# Autodesk Inventor assembly: Refined Glock
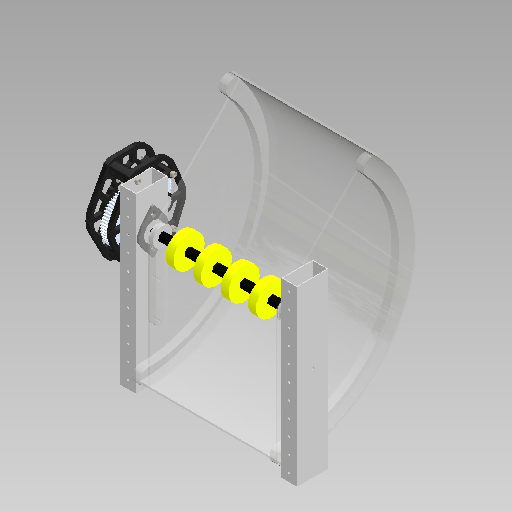
[picture p0: Inventor's stored thumbnail of the model, 512x512]
Saved by Autodesk Inventor 2021 (Build 250183000, 183)
## iProperties
Created: 2021-02-04
Part Number: Refined Glock
Document SubType Name: Assembly
Designer: aidan
Author: aidan
## Documents named in this file (12)
- C:\Users\Merkileg\Documents\t3-cad\CAD\2021 Specific Parts\Refined Glock.iam
- C:\Users\Merkileg\Documents\t3-cad\CAD\2021 Specific Parts\Curved Lexan Support.ipt
- C:\Users\Merkileg\Documents\t3-cad\CAD\2021 Specific Parts\Shooter side panel.ipt
- C:\Users\Merkileg\Documents\t3-cad\CAD\2021 Specific Parts\Lexan Glock Back.ipt
- C:\Users\Merkileg\Documents\t3-cad\CAD\Bearing for THUNDER.ipt
- C:\Users\Merkileg\Documents\t3-cad\CAD\WCP SS_Shrinkwrap.ipt
- C:\Users\Merkileg\Documents\t3-cad\CAD\2021 Specific Parts\VersaFrame Support for Glock.ipt
- C:\Users\Merkileg\Documents\t3-cad\CAD\Drive Train CAD\WCP DS Gearbox\WCP Gearbox Mount.ipt
- C:\Users\Merkileg\Documents\t3-cad\CAD\2021 Specific Parts\Side lexan spacer for Glock.ipt
- C:\Users\Merkileg\Documents\t3-cad\CAD\Generic and Stock\11.75in THUNDERSHAFT.ipt
- C:\Users\Merkileg\Documents\t3-cad\CAD\Tristan's CAD\Glock\2 in Compliance Wheel.ipt
- C:\Users\Merkileg\Documents\t3-cad\CAD\2021 Specific Parts\VerseFrame 11in w hole.ipt
## Components (19 placed, 11 different names)
1. Curved Lexan Support:1 — Mate:3, Mate:5, Mate:6, Mate:14
2. Curved Lexan Support:2 — Mate:3, Mate:4, Mate:5, Mate:7, Flush:3, Mate:9
3. Shooter side panel:1 — Flush:1, Flush:2, Mate:6, Mate:8, Mate:10, Mate:12, Angle:1, Mate:35
4. Shooter side panel:2 — Flush:1, Flush:2, Mate:4, Mate:7, Mate:8, Flush:4, Mate:11, Mate:13, Mate:30
5. Lexan Glock Back:1 — Flush:3, Mate:9, Flush:4
6. Bearing for THUNDER:1 — Mate:11, Mate:13, Flush:5, Mate:32, Flush:12
7. Bearing for THUNDER:2 — Mate:10, Mate:12, Flush:5, Mate:15, Mate:21, Mate:31
8. WCP SS_Shrinkwrap:1 — Mate:21, Mate:22, Angle:2
9. VersaFrame Support for Glock:1 — Mate:14, Mate:15, Angle:1, Mate:16, Mate:17, Mate:18, Mate:22, Angle:2, Flush:9, Mate:27, Flush:10, Flush:11
10. WCP Gearbox Mount:1 — Mate:16, Mate:17, Mate:18, Mate:19, Mate:20
11. Bearing for THUNDER:3 — Mate:19, Mate:20
12. Side lexan spacer for Glock:1 — Flush:8, Mate:26, Flush:9, Mate:27
13. Side lexan spacer for Glock:2 — Flush:8, Mate:26, Mate:28, Mate:29, Mate:30
14. VerseFrame 11in w hole:1 — Mate:28, Flush:10, Flush:11, Mate:29
15. 11.75in THUNDERSHAFT:1 — Mate:31, Mate:32, Flush:12, Mate:33, Mate:34
16. 2 in Compliance Wheel:1 — Flush:14, Flush:15, Flush:16, Flush:17, Flush:18, Mate:35, Mate:36
17. 2 in Compliance Wheel:2 — Flush:15, Flush:16, Mate:34, Mate:38
18. 2 in Compliance Wheel:3 — Flush:13, Flush:18, Mate:33, Mate:37, Mate:38
19. 2 in Compliance Wheel:4 — Flush:13, Flush:14, Flush:17, Mate:36, Mate:37
## Relationships (51: Mate 33, Flush 16, Angle 2)
- Flush:1: Shooter side panel:1 ↔ Shooter side panel:2
- Flush:2: Shooter side panel:1 ↔ Shooter side panel:2
- Mate:3: Curved Lexan Support:1 ↔ Curved Lexan Support:2
- Mate:4: Curved Lexan Support:2 ↔ Shooter side panel:2
- Mate:5: Curved Lexan Support:1 ↔ Curved Lexan Support:2
- Mate:6: Curved Lexan Support:1 ↔ Shooter side panel:1
- Mate:7: Curved Lexan Support:2 ↔ Shooter side panel:2
- Mate:8 (203.2 mm): Shooter side panel:1 ↔ Shooter side panel:2
- Flush:3: Curved Lexan Support:2 ↔ Lexan Glock Back:1
- Mate:9: Curved Lexan Support:2 ↔ Lexan Glock Back:1
- Flush:4: Shooter side panel:2 ↔ Lexan Glock Back:1
- Mate:10: Shooter side panel:1 ↔ Bearing for THUNDER:2
- Mate:11: Shooter side panel:2 ↔ Bearing for THUNDER:1
- Mate:12: Shooter side panel:1 ↔ Bearing for THUNDER:2
- Mate:13: Shooter side panel:2 ↔ Bearing for THUNDER:1
- Flush:5: Bearing for THUNDER:1 ↔ Bearing for THUNDER:2
- Mate:14: Curved Lexan Support:1 ↔ VersaFrame Support for Glock:1
- Mate:15: Bearing for THUNDER:2 ↔ VersaFrame Support for Glock:1
- Angle:1 (0 deg): Shooter side panel:1 ↔ VersaFrame Support for Glock:1
- Mate:16: VersaFrame Support for Glock:1 ↔ WCP Gearbox Mount:1
- Mate:17: VersaFrame Support for Glock:1 ↔ WCP Gearbox Mount:1
- Mate:18: VersaFrame Support for Glock:1 ↔ WCP Gearbox Mount:1
- Mate:19: WCP Gearbox Mount:1 ↔ Bearing for THUNDER:3
- Mate:20: WCP Gearbox Mount:1 ↔ Bearing for THUNDER:3
- Mate:21: Bearing for THUNDER:2 ↔ WCP SS_Shrinkwrap:1
- Mate:22: WCP SS_Shrinkwrap:1 ↔ VersaFrame Support for Glock:1
- Angle:2 (0 deg): WCP SS_Shrinkwrap:1 ↔ VersaFrame Support for Glock:1
- Flush:8: Side lexan spacer for Glock:1 ↔ Side lexan spacer for Glock:2
- Mate:26: Side lexan spacer for Glock:1 ↔ Side lexan spacer for Glock:2
- Flush:9 (-19.05 mm): VersaFrame Support for Glock:1 ↔ Side lexan spacer for Glock:1
- Mate:27: VersaFrame Support for Glock:1 ↔ Side lexan spacer for Glock:1
- Mate:28: Side lexan spacer for Glock:2 ↔ VerseFrame 11in w hole:1
- Flush:10: VersaFrame Support for Glock:1 ↔ VerseFrame 11in w hole:1
- Flush:11: VersaFrame Support for Glock:1 ↔ VerseFrame 11in w hole:1
- Mate:29: Side lexan spacer for Glock:2 ↔ VerseFrame 11in w hole:1
- Mate:30: Shooter side panel:2 ↔ Side lexan spacer for Glock:2
- Mate:31: Bearing for THUNDER:2 ↔ 11.75in THUNDERSHAFT:1
- Mate:32: Bearing for THUNDER:1 ↔ 11.75in THUNDERSHAFT:1
- Flush:12 (-6.35 mm): Bearing for THUNDER:1 ↔ 11.75in THUNDERSHAFT:1
- Flush:13: 2 in Compliance Wheel:3 ↔ 2 in Compliance Wheel:4
- Flush:14: 2 in Compliance Wheel:1 ↔ 2 in Compliance Wheel:4
- Flush:15: 2 in Compliance Wheel:1 ↔ 2 in Compliance Wheel:2
- Flush:16: 2 in Compliance Wheel:1 ↔ 2 in Compliance Wheel:2
- Flush:17: 2 in Compliance Wheel:1 ↔ 2 in Compliance Wheel:4
- Flush:18: 2 in Compliance Wheel:1 ↔ 2 in Compliance Wheel:3
- Mate:33: 11.75in THUNDERSHAFT:1 ↔ 2 in Compliance Wheel:3
- Mate:34: 11.75in THUNDERSHAFT:1 ↔ 2 in Compliance Wheel:2
- Mate:35 (31.75 mm): Shooter side panel:1 ↔ 2 in Compliance Wheel:1
- Mate:36 (31.75 mm): 2 in Compliance Wheel:1 ↔ 2 in Compliance Wheel:4
- Mate:37 (31.75 mm): 2 in Compliance Wheel:3 ↔ 2 in Compliance Wheel:4
- Mate:38 (31.75 mm): 2 in Compliance Wheel:2 ↔ 2 in Compliance Wheel:3
